# Autodesk Inventor assembly: Vibrometer Cover
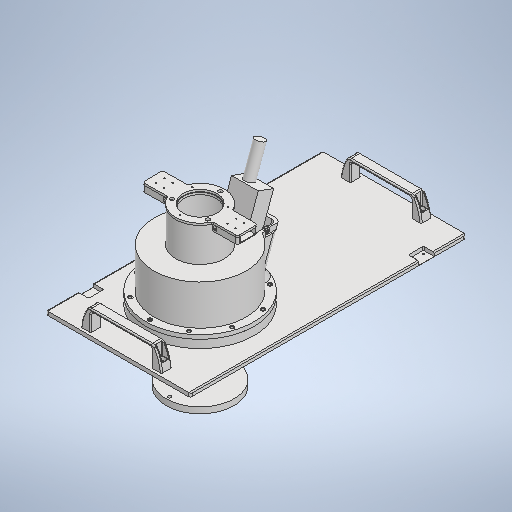
[picture p0: Inventor's stored thumbnail of the model, 512x512]
Saved by Autodesk Inventor 2026.2 (Build 302298000, 298)
## iProperties
Created: 2026-03-30
Part Number: Vibrometer Cover
Document SubType Name: Assembly
Designer: mumin
Author: mumin
## Documents named in this file (10)
- C:\GitHub\In-situ-monitoring-of-powder-bed-fusion-additive-manufacturing\system_development\Orichalcum\v0.4\Vibrometer Cover.iam
- C:\GitHub\In-situ-monitoring-of-powder-bed-fusion-additive-manufacturing\system_development\Orichalcum\v0.4\12mm Cover.ipt
- C:\GitHub\In-situ-monitoring-of-powder-bed-fusion-additive-manufacturing\system_development\Orichalcum\v0.4\Handle.ipt
- C:\GitHub\In-situ-monitoring-of-powder-bed-fusion-additive-manufacturing\system_development\Orichalcum\v0.4\SealedGlassRing.ipt
- C:\GitHub\In-situ-monitoring-of-powder-bed-fusion-additive-manufacturing\system_development\Orichalcum\v0.4\Vibrometer Housing.ipt
- C:\GitHub\In-situ-monitoring-of-powder-bed-fusion-additive-manufacturing\system_development\Orichalcum\v0.4\Build Plate.ipt
- C:\GitHub\In-situ-monitoring-of-powder-bed-fusion-additive-manufacturing\system_development\Orichalcum\v0.4\Updated Laser Scanner.ipt
- C:\GitHub\In-situ-monitoring-of-powder-bed-fusion-additive-manufacturing\system_development\Orichalcum\v0.4\Mithril Center Cylinder.ipt
- C:\GitHub\In-situ-monitoring-of-powder-bed-fusion-additive-manufacturing\system_development\Orichalcum\v0.4\Metal Head Plate.ipt
- C:\GitHub\In-situ-monitoring-of-powder-bed-fusion-additive-manufacturing\system_development\Orichalcum\v0.4\Head Plate Insert.ipt
## Components (11 placed, 9 different names)
1. 12mm Cover:1 — Insert:1, Insert:2, Insert:3, Insert:4, Insert:7
2. Handle:1 — Insert:1
3. Handle:2 — Insert:2
4. SealedGlassRing:1 — Insert:3, Insert:4, Insert:5, Insert:6
5. Vibrometer Housing:1 — Insert:5, Insert:6, Cylindrical:1, Mate:1, Mate:2
6. Build Plate:1 — Insert:7
7. Updated Laser Scanner:1 — Mate:1, Mate:2
8. Mithril Center Cylinder:1 — Cylindrical:1, Insert:8, Insert:9
9. Metal Head Plate:1 — Insert:8, Insert:9, Insert:10, Flush:1, Insert:11, Flush:2
10. Head Plate Insert:1 — Insert:10, Flush:1
11. Head Plate Insert:2 — Insert:11, Flush:2
## Relationships (16: Insert 11, Mate 2, Flush 2, CylindricalJoint 1)
- Insert:1: 12mm Cover:1 ↔ Handle:1
- Insert:2: 12mm Cover:1 ↔ Handle:2
- Insert:3: 12mm Cover:1 ↔ SealedGlassRing:1
- Insert:4: 12mm Cover:1 ↔ SealedGlassRing:1
- Insert:5: SealedGlassRing:1 ↔ Vibrometer Housing:1
- Insert:6: SealedGlassRing:1 ↔ Vibrometer Housing:1
- Insert:7 (150 mm): 12mm Cover:1 ↔ Build Plate:1
- Cylindrical:1: Vibrometer Housing:1 ↔ Mithril Center Cylinder:1
- Mate:1 (15.5 mm): Vibrometer Housing:1 ↔ Updated Laser Scanner:1
- Mate:2 (12 mm): Vibrometer Housing:1 ↔ Updated Laser Scanner:1
- Insert:8: Mithril Center Cylinder:1 ↔ Metal Head Plate:1
- Insert:9: Mithril Center Cylinder:1 ↔ Metal Head Plate:1
- Insert:10: Metal Head Plate:1 ↔ Head Plate Insert:1
- Flush:1: Metal Head Plate:1 ↔ Head Plate Insert:1
- Insert:11: Metal Head Plate:1 ↔ Head Plate Insert:2
- Flush:2: Metal Head Plate:1 ↔ Head Plate Insert:2
